# Autodesk Inventor assembly: Cockpit_
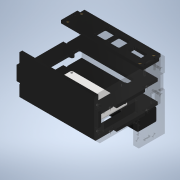
[picture p0: Inventor's stored thumbnail of the model, 180x180]
Saved by Autodesk Inventor 2020.4 (Build 244396000, 396)
## iProperties
Created: 2022-01-06
Part Number: Cockpit_
Document SubType Name: Assembly
Designer: Masato Kubotera
Mass: 586.569 g
Surface Area: 2053.33 cm^2
Volume: 316.504 cm^3
Density: 1.85327 g/cm^3
Author: Masato Kubotera
## Documents named in this file (10)
- C:\Users\Masato\Documents\Inventor\CIT Brains_Inventor\OpenPlatform_ver3_0\UpperBody\Cockpit\Cockpit_.iam
- C:\Users\Masato\Documents\Inventor\CIT Brains_Inventor\OpenPlatform_ver3_0\UpperBody\Cockpit\Cockpit_side_frame.ipt
- C:\Users\Masato\Documents\Inventor\CIT Brains_Inventor\OpenPlatform_ver3_0\UpperBody\Cockpit\Cockpit_front_frame.ipt
- C:\Users\Masato\Documents\Inventor\CIT Brains_Inventor\OpenPlatform_ver3_0\UpperBody\Cockpit\Cockpit_bottom_frame.ipt
- C:\Users\Masato\Documents\Inventor\CIT Brains_Inventor\OpenPlatform_ver3_0\UpperBody\Cockpit\Cockpit_middle_frame.ipt
- C:\Users\Masato\Documents\Inventor\CIT Brains_Inventor\OpenPlatform_ver3_0\UpperBody\Cockpit\MainBoard.ipt
- C:\Users\Masato\Documents\Inventor\CIT Brains_Inventor\OpenPlatform_ver3_0\ReadyMade\Battery\HP-G830C2800S3.ipt
- C:\Users\Masato\Documents\Inventor\CIT Brains_Inventor\OpenPlatform_ver3_0\UpperBody\Cockpit\Cockpit_top_frame.ipt
- C:\Users\Masato\Documents\Inventor\CIT Brains_Inventor\OpenPlatform_ver3_0\UpperBody\Cockpit\Cockpit_back_frame.ipt
- C:\Users\Masato\Documents\Inventor\CIT Brains_Inventor\OpenPlatform_ver3_0\ReadyMade\InsertNut\UD-43040.ipt
## Components (12 placed, 9 different names)
1. Cockpit_side_frame:1 — 挿入:1, 挿入:2, 挿入:3, 挿入:4, 挿入:5, 挿入:6, フラッシュ:1, メイト:1, フラッシュ:2, フラッシュ:3, 挿入:13, 挿入:14, 挿入:15, 挿入:16
2. Cockpit_front_frame:1 — 挿入:1, 挿入:2
3. Cockpit_bottom_frame:1 — 挿入:3, 挿入:4, 挿入:9, 挿入:10
4. Cockpit_middle_frame:1 — 挿入:5, 挿入:6
5. MainBoard:1 — 挿入:9, 挿入:10
6. HP-G830C2800S3:1 — フラッシュ:3
7. Cockpit_top_frame:1 — 挿入:13, 挿入:14, 挿入:17, 挿入:18, 挿入:19, 挿入:20
8. Cockpit_back_frame:1 — 挿入:15, 挿入:16
9. UD-43040:1 — 挿入:17
10. UD-43040:2 — 挿入:18
11. UD-43040:3 — 挿入:19
12. UD-43040:4 — 挿入:20
## Relationships (20: Insert 16, Flush 3, Mate 1)
- 挿入:1 [Insert]: Cockpit_side_frame:1 ↔ Cockpit_front_frame:1
- 挿入:2 [Insert]: Cockpit_side_frame:1 ↔ Cockpit_front_frame:1
- 挿入:3 [Insert]: Cockpit_side_frame:1 ↔ Cockpit_bottom_frame:1
- 挿入:4 [Insert]: Cockpit_side_frame:1 ↔ Cockpit_bottom_frame:1
- 挿入:5 [Insert]: Cockpit_side_frame:1 ↔ Cockpit_middle_frame:1
- 挿入:6 [Insert]: Cockpit_side_frame:1 ↔ Cockpit_middle_frame:1
- フラッシュ:1 [Flush]: Cockpit_side_frame:1
- メイト:1 [Mate]: Cockpit_side_frame:1
- フラッシュ:2 [Flush]: Cockpit_side_frame:1
- 挿入:9 [Insert] (5 mm): Cockpit_bottom_frame:1 ↔ MainBoard:1
- 挿入:10 [Insert] (5 mm): Cockpit_bottom_frame:1 ↔ MainBoard:1
- フラッシュ:3 [Flush] (-5 mm): Cockpit_side_frame:1 ↔ HP-G830C2800S3:1
- 挿入:13 [Insert]: Cockpit_side_frame:1 ↔ Cockpit_top_frame:1
- 挿入:14 [Insert]: Cockpit_side_frame:1 ↔ Cockpit_top_frame:1
- 挿入:15 [Insert]: Cockpit_side_frame:1 ↔ Cockpit_back_frame:1
- 挿入:16 [Insert]: Cockpit_side_frame:1 ↔ Cockpit_back_frame:1
- 挿入:17 [Insert]: Cockpit_top_frame:1 ↔ UD-43040:1
- 挿入:18 [Insert]: Cockpit_top_frame:1 ↔ UD-43040:2
- 挿入:19 [Insert]: Cockpit_top_frame:1 ↔ UD-43040:3
- 挿入:20 [Insert]: Cockpit_top_frame:1 ↔ UD-43040:4
